# Autodesk Inventor assembly: OBG-Oberbau
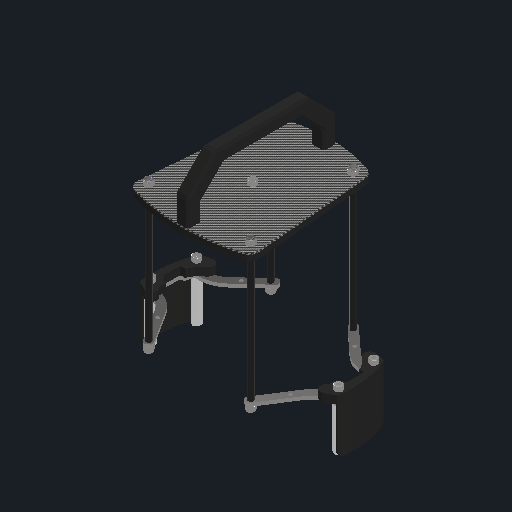
[picture p0: Inventor's stored thumbnail of the model, 512x512]
Saved by Autodesk Inventor 2025.2 (Build 292293000, 293)
## iProperties
Created: 2024-11-26
Part Number: OBG-Oberbau
Document SubType Name: Assembly
Designer: Fabian
Author: Fabian
## Documents named in this file (15)
- C:\Users\Faabs\Desktop\HBG v2025\Oberbaugruppen\OBG-Oberbau\OBG-Oberbau.iam
- C:\Users\Faabs\Desktop\HBG v2025\Oberbaugruppen\OBG-Oberbau\Bauteile\Spiegelhalterung.ipt
- C:\Users\Faabs\Desktop\HBG v2025\Oberbaugruppen\OBG-Oberbau\Bauteile\Gewindestange.ipt
- C:\Users\Faabs\Desktop\HBG v2025\Oberbaugruppen\OBG-Oberbau\Bauteile\Schwungstrebe.ipt
- C:\Users\Faabs\Desktop\HBG v2025\Oberbaugruppen\OBG-Oberbau\Bauteile\M4 Sicherungsmutter.ipt
- C:\Users\Faabs\Desktop\HBG v2025\Oberbaugruppen\OBG-Oberbau\Bauteile\Abstandsbolzen 38mm.ipt
- C:\Users\Faabs\Desktop\HBG v2025\Oberbaugruppen\OBG-Oberbau\Bauteile\CarbonRohr.ipt
- C:\Users\Faabs\Desktop\HBG v2025\Verbindungselemente\DIN 912\DIN 912 - M4 x 0,7 x 8 x 6,25.ipt
- C:\Users\Faabs\Desktop\HBG v2025\Oberbaugruppen\OBG-Oberbau\Bauteile\Spiegel.ipt
- C:\Users\Faabs\Desktop\HBG v2025\Oberbaugruppen\OBG-Oberbau\Bauteile\Griff.ipt
- C:\Users\Faabs\Desktop\HBG v2025\Verbindungselemente\DIN 7984\DIN 7984 - M3 x 5.ipt
- C:\Users\Faabs\Desktop\HBG v2025\Oberbaugruppen\OBG-Oberbau\Bauteile\Spiegelabdeckung.ipt
- C:\Users\Faabs\Desktop\HBG v2025\Oberbaugruppen\OBG-Oberbau\Bauteile\Abdeckung.ipt
- C:\Users\Faabs\Desktop\HBG v2025\Oberbaugruppen\OBG-Oberbau\Bauteile\SpiegelabdeckungSSL.ipt
- C:\Users\Faabs\Desktop\HBG v2025\Oberbaugruppen\OBG-Oberbau\Bauteile\Abdeckung_MIR.ipt
## Components (36 placed, 14 different names)
1. Spiegelhalterung:1 — Passend:1, Passend:2, Passend:5, Passend:6, Fluchtend:2, Fluchtend:3, Passend:17, Passend:18, Passend:19, Passend:20, Passend:40, Passend:41, Einfügen:11, Passend:44, Einfügen:14, Einfügen:15, Passend:47, Passend:56
2. Schwungstrebe:1 — Passend:7, Passend:8, Passend:21, Einfügen:1, Einfügen:2, Passend:28, Passend:29, Passend:34, Passend:35, Fluchtend:5, Passend:48, Passend:50, Fluchtend:8, Fluchtend:9
3. Schwungstrebe:2 — Passend:36, Passend:37, Fluchtend:5, Passend:38, Passend:39, Einfügen:9, Einfügen:10, Fluchtend:6, Fluchtend:7, Passend:58, Passend:59, Passend:60
4. Spiegel:1 — Passend:40, Passend:41, Passend:46
5. Griff:1 — Passend:44, Einfügen:14, Einfügen:15
6. Spiegelabdeckung:1 — Passend:45, Passend:46, Passend:47, Einfügen:16, Einfügen:17
7. Abdeckung:2 — Passend:48, Passend:49, Passend:50, Einfügen:20, Einfügen:21
8. Abdeckung_MIR:1 — Passend:58, Passend:59, Passend:60, Einfügen:22, Einfügen:23
9. SpiegelabdeckungSSL:1 — Passend:54, Passend:55, Passend:56
10. DIN 7984 M3 x 5:2 — Einfügen:16
11. DIN 7984 M3 x 5:1 — Einfügen:17
12. DIN 912 - ersetzt durch DIN EN ISO 4762 M4 x 8:5 — Einfügen:11, Passend:54
13. M4 Sicherungsmutter:1 — Passend:14, Passend:19
14. M4 Sicherungsmutter:2 — Passend:16, Passend:17
15. M4 Sicherungsmutter:3 — Passend:15, Passend:20
16. M4 Sicherungsmutter:4 — Passend:13, Passend:18, Fluchtend:4
17. M4 Sicherungsmutter:5 — Passend:22, Passend:28, Fluchtend:9
18. M4 Sicherungsmutter:6 — Passend:24, Passend:38, Fluchtend:6
19. M4 Sicherungsmutter:7 — Passend:23, Passend:29, Fluchtend:8
20. M4 Sicherungsmutter:8 — Passend:25, Passend:39, Fluchtend:7
21. DIN 912 - ersetzt durch DIN EN ISO 4762 M4 x 8:1 — Einfügen:20
22. DIN 912 - ersetzt durch DIN EN ISO 4762 M4 x 8:2 — Einfügen:21
23. DIN 912 - ersetzt durch DIN EN ISO 4762 M4 x 8:3 — Einfügen:23
24. DIN 912 - ersetzt durch DIN EN ISO 4762 M4 x 8:4 — Einfügen:22
25. Abstandsbolzen 38mm:1 — Einfügen:1, Passend:49
26. Abstandsbolzen 38mm:2 — Einfügen:2
27. Abstandsbolzen 38mm:3 — Einfügen:10
28. Abstandsbolzen 38mm:4 — Einfügen:9
29. Gewindestange:1 — Passend:2, Passend:7, Passend:11, Passend:14, Passend:23, Passend:31
30. Gewindestange:2 — Passend:1, Passend:8, Passend:9, Passend:13, Fluchtend:4, Passend:22, Passend:30
31. Gewindestange:3 — Passend:5, Passend:10, Passend:16, Passend:24, Passend:32, Passend:45
32. Gewindestange:4 — Passend:6, Passend:12, Passend:15, Passend:25, Passend:33
33. CarbonRohr:1 — Passend:30, Passend:34, Passend:55
34. CarbonRohr:2 — Passend:33, Passend:37
35. CarbonRohr:3 — Passend:32, Passend:36
36. CarbonRohr:4 — Passend:31, Passend:35
## Relationships (71: Mate 50, Insert 13, Flush 8)
- Passend:1 [Mate]: Spiegelhalterung:1 ↔ Gewindestange:2
- Passend:2 [Mate]: Spiegelhalterung:1 ↔ Gewindestange:1
- Passend:5 [Mate]: Spiegelhalterung:1 ↔ Gewindestange:3
- Passend:6 [Mate]: Spiegelhalterung:1 ↔ Gewindestange:4
- Passend:7 [Mate]: Schwungstrebe:1 ↔ Gewindestange:1
- Passend:8 [Mate]: Schwungstrebe:1 ↔ Gewindestange:2
- Passend:9 [Mate] (32 mm): Gewindestange:2
- Passend:10 [Mate] (32 mm): Gewindestange:3
- Passend:11 [Mate] (32 mm): Gewindestange:1
- Passend:12 [Mate] (32 mm): Gewindestange:4
- Fluchtend:2 [Flush]: Spiegelhalterung:1
- Fluchtend:3 [Flush]: Spiegelhalterung:1
- Passend:13 [Mate]: M4 Sicherungsmutter:4 ↔ Gewindestange:2
- Passend:14 [Mate]: M4 Sicherungsmutter:1 ↔ Gewindestange:1
- Passend:15 [Mate]: M4 Sicherungsmutter:3 ↔ Gewindestange:4
- Passend:16 [Mate]: M4 Sicherungsmutter:2 ↔ Gewindestange:3
- Passend:17 [Mate]: Spiegelhalterung:1 ↔ M4 Sicherungsmutter:2
- Passend:18 [Mate]: Spiegelhalterung:1 ↔ M4 Sicherungsmutter:4
- Passend:19 [Mate]: Spiegelhalterung:1 ↔ M4 Sicherungsmutter:1
- Passend:20 [Mate]: Spiegelhalterung:1 ↔ M4 Sicherungsmutter:3
- Fluchtend:4 [Flush] (-0.5 mm): M4 Sicherungsmutter:4 ↔ Gewindestange:2
- Passend:21 [Mate] (38 mm): Schwungstrebe:1
- Einfügen:1 [Insert]: Schwungstrebe:1 ↔ Abstandsbolzen 38mm:1
- Einfügen:2 [Insert]: Schwungstrebe:1 ↔ Abstandsbolzen 38mm:2
- Passend:22 [Mate]: M4 Sicherungsmutter:5 ↔ Gewindestange:2
- Passend:23 [Mate]: M4 Sicherungsmutter:7 ↔ Gewindestange:1
- Passend:24 [Mate]: M4 Sicherungsmutter:6 ↔ Gewindestange:3
- Passend:25 [Mate]: M4 Sicherungsmutter:8 ↔ Gewindestange:4
- Passend:28 [Mate]: Schwungstrebe:1 ↔ M4 Sicherungsmutter:5
- Passend:29 [Mate]: Schwungstrebe:1 ↔ M4 Sicherungsmutter:7
- Passend:30 [Mate]: Gewindestange:2 ↔ CarbonRohr:1
- Passend:31 [Mate]: Gewindestange:1 ↔ CarbonRohr:4
- Passend:32 [Mate]: Gewindestange:3 ↔ CarbonRohr:3
- Passend:33 [Mate]: Gewindestange:4 ↔ CarbonRohr:2
- Passend:34 [Mate]: Schwungstrebe:1 ↔ CarbonRohr:1
- Passend:35 [Mate]: Schwungstrebe:1 ↔ CarbonRohr:4
- Passend:36 [Mate]: Schwungstrebe:2 ↔ CarbonRohr:3
- Passend:37 [Mate]: Schwungstrebe:2 ↔ CarbonRohr:2
- Fluchtend:5 [Flush]: Schwungstrebe:1 ↔ Schwungstrebe:2
- Passend:38 [Mate]: Schwungstrebe:2 ↔ M4 Sicherungsmutter:6
- Passend:39 [Mate]: Schwungstrebe:2 ↔ M4 Sicherungsmutter:8
- Einfügen:9 [Insert]: Schwungstrebe:2 ↔ Abstandsbolzen 38mm:4
- Einfügen:10 [Insert]: Schwungstrebe:2 ↔ Abstandsbolzen 38mm:3
- Passend:40 [Mate]: Spiegelhalterung:1 ↔ Spiegel:1
- Passend:41 [Mate]: Spiegelhalterung:1 ↔ Spiegel:1
- Einfügen:11 [Insert]: Spiegelhalterung:1 ↔ DIN 912 - ersetzt durch DIN EN ISO 4762 M4 x 8:5
- Passend:44 [Mate]: Spiegelhalterung:1 ↔ Griff:1
- Einfügen:14 [Insert]: Spiegelhalterung:1 ↔ Griff:1
- Einfügen:15 [Insert]: Spiegelhalterung:1 ↔ Griff:1
- Passend:45 [Mate]: Spiegelabdeckung:1 ↔ Gewindestange:3
- Passend:46 [Mate]: Spiegel:1 ↔ Spiegelabdeckung:1
- Passend:47 [Mate]: Spiegelhalterung:1 ↔ Spiegelabdeckung:1
- Einfügen:16 [Insert]: Spiegelabdeckung:1 ↔ DIN 7984 M3 x 5:2
- Einfügen:17 [Insert]: Spiegelabdeckung:1 ↔ DIN 7984 M3 x 5:1
- Passend:48 [Mate]: Schwungstrebe:1 ↔ Abdeckung:2
- Passend:49 [Mate]: Abdeckung:2 ↔ Abstandsbolzen 38mm:1
- Passend:50 [Mate]: Schwungstrebe:1 ↔ Abdeckung:2
- Passend:54 [Mate]: SpiegelabdeckungSSL:1 ↔ DIN 912 - ersetzt durch DIN EN ISO 4762 M4 x 8:5
- Passend:55 [Mate]: SpiegelabdeckungSSL:1 ↔ CarbonRohr:1
- Passend:56 [Mate]: Spiegelhalterung:1 ↔ SpiegelabdeckungSSL:1
- Fluchtend:6 [Flush] (0.05 mm): Schwungstrebe:2 ↔ M4 Sicherungsmutter:6
- Fluchtend:7 [Flush] (0.05 mm): Schwungstrebe:2 ↔ M4 Sicherungsmutter:8
- Fluchtend:8 [Flush] (0.05 mm): Schwungstrebe:1 ↔ M4 Sicherungsmutter:7
- Fluchtend:9 [Flush] (0.05 mm): Schwungstrebe:1 ↔ M4 Sicherungsmutter:5
- Einfügen:20 [Insert]: Abdeckung:2 ↔ DIN 912 - ersetzt durch DIN EN ISO 4762 M4 x 8:1
- Einfügen:21 [Insert]: Abdeckung:2 ↔ DIN 912 - ersetzt durch DIN EN ISO 4762 M4 x 8:2
- Passend:58 [Mate]: Schwungstrebe:2 ↔ Abdeckung_MIR:1
- Passend:59 [Mate]: Schwungstrebe:2 ↔ Abdeckung_MIR:1
- Passend:60 [Mate]: Schwungstrebe:2 ↔ Abdeckung_MIR:1
- Einfügen:22 [Insert]: Abdeckung_MIR:1 ↔ DIN 912 - ersetzt durch DIN EN ISO 4762 M4 x 8:4
- Einfügen:23 [Insert]: Abdeckung_MIR:1 ↔ DIN 912 - ersetzt durch DIN EN ISO 4762 M4 x 8:3
